# Autodesk Inventor assembly: Oven Control
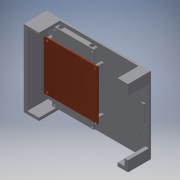
[picture p0: Inventor's stored thumbnail of the model, 180x180]
Saved by Autodesk Inventor 2019 (Build 230136000, 136)
## iProperties
Created: 2019-03-10
Part Number: Oven Control
Document SubType Name: Assembly
Designer: savo
Author: savo
## Documents named in this file (5)
- C:\OneDrive\OneDrive - University of Toronto\HPVDT\Oven\CAD Files\Oven Control.iam
- C:\OneDrive\OneDrive - University of Toronto\HPVDT\Oven\CAD Files\Keypad.ipt
- C:\OneDrive\OneDrive - University of Toronto\HPVDT\Oven\CAD Files\LCD Screen.ipt
- C:\OneDrive\OneDrive - University of Toronto\HPVDT\Oven\CAD Files\PCB.ipt
- C:\OneDrive\OneDrive - University of Toronto\HPVDT\Oven\CAD Files\Case.ipt
## Components (4 placed, 4 different names)
1. Keypad:1 — Flush:1, Flush:2, Mate:1, Mate:3, Mate:4, Flush:3
2. LCD Screen:1 — Flush:1, Mate:1, Mate:2, Mate:3, Flush:4
3. PCB:1 — Mate:2, Mate:4, Flush:4
4. Case:1 — Flush:3
## Relationships (8: Flush 4, Mate 4)
- Flush:1: Keypad:1 ↔ LCD Screen:1
- Flush:2: Keypad:1
- Mate:1 (8 mm): Keypad:1 ↔ LCD Screen:1
- Mate:2 (3 mm): LCD Screen:1 ↔ PCB:1
- Mate:3 (8 mm): Keypad:1 ↔ LCD Screen:1
- Mate:4: Keypad:1 ↔ PCB:1
- Flush:3: Keypad:1 ↔ Case:1
- Flush:4 (10 mm): LCD Screen:1 ↔ PCB:1
